# Autodesk Inventor assembly: wheel
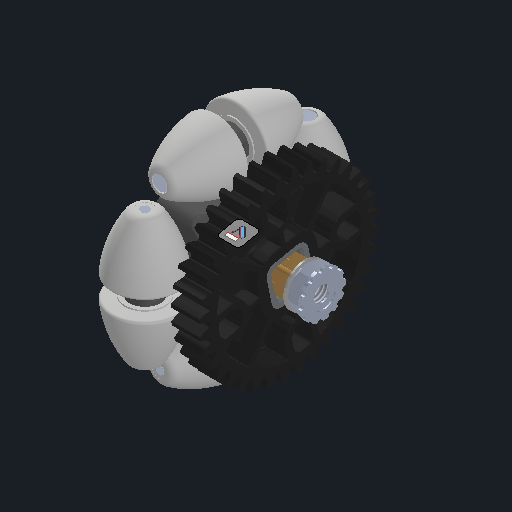
[picture p0: Inventor's stored thumbnail of the model, 512x512]
Saved by Autodesk Inventor 2025 (Build 290162000, 162)
## iProperties
Created: 2024-10-11
Part Number: wheel
Document SubType Name: Assembly
Designer: Averey Ku
Author: Averey Ku
## Documents named in this file (7)
- D:\vex_robotics_high_stakes\hardware\cad\bots\high_stakes_v2\chassis_v2\drivebay\wheel.iam
- D:\vex_robotics_high_stakes\hardware\cad\robpros_cad_lib\Motion\Wheels\Omni Wheel\2.00 Omni AS, No Insert.ipt
- D:\vex_robotics_high_stakes\hardware\cad\robpros_cad_lib\Modified Parts\modified_parts\Half Cut HS 36T Gear, No Insert.ipt
- D:\vex_robotics_high_stakes\hardware\cad\robpros_cad_lib\Motion\HS Shaft Adapter Circle.ipt
- D:\vex_robotics_high_stakes\hardware\cad\robpros_cad_lib\Structure\Hardware\Nut Keps.ipt
- D:\vex_robotics_high_stakes\hardware\cad\robpros_cad_lib\Motion\Spacers\Washer Steel\SWasher .375 OD x .015625.ipt
- D:\vex_robotics_high_stakes\hardware\cad\robpros_cad_lib\Motion\Spacers\Washer Steel.ipt
## Components (7 placed, 5 different names)
1. Half Cut HS 36T Gear, No Insert:1 — Insert:13
2. HS Shaft Adapter Circle:1 — Insert:8, Insert:11
3. Nut Keps:1 — Mate:1, Insert:9
4. SWasher .375 OD x .015625:2 — Insert:11, Insert:12
5. 2.00 Omni AS, No Insert:1 — Insert:12, Insert:13
6. SWasher .375 OD x .015625:3 — Insert:9, Insert:10
7. HS Shaft Adapter Circle:2 — Insert:8, Insert:10
## Relationships (8: Insert 6, Angle 1, Mate 1)
- [Angle] (0 deg): Half Cut HS 36T Gear, No Insert:1 ↔ HS Shaft Adapter Circle:1
- Mate:1: Nut Keps:1
- Insert:8: HS Shaft Adapter Circle:1 ↔ HS Shaft Adapter Circle:2
- Insert:9: Nut Keps:1 ↔ SWasher .375 OD x .015625:3
- Insert:10: SWasher .375 OD x .015625:3 ↔ HS Shaft Adapter Circle:2
- Insert:11: HS Shaft Adapter Circle:1 ↔ SWasher .375 OD x .015625:2
- Insert:12: SWasher .375 OD x .015625:2 ↔ 2.00 Omni AS, No Insert:1
- Insert:13: Half Cut HS 36T Gear, No Insert:1 ↔ 2.00 Omni AS, No Insert:1
